# Autodesk Inventor assembly: Zed Kicker
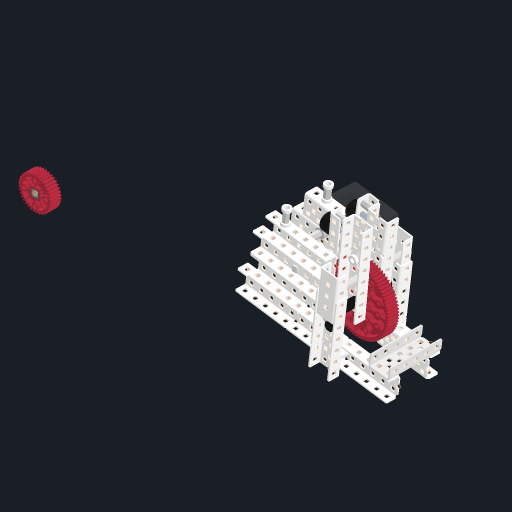
[picture p0: Inventor's stored thumbnail of the model, 512x512]
Saved by Autodesk Inventor 2023.2 (Build 272271030, 271C)
## iProperties
Created: 2024-02-14
Part Number: Zed Kicker
Document SubType Name: Assembly
Designer: Michael
Author: Michael
## Documents named in this file (35)
- C:\Users\black\OneDrive\Pictures\Documents\GitHub\New folder\2024-599Z\Cad\NEW Kicker\Zed Kicker.iam
- C:\Users\black\OneDrive\Pictures\Documents\GitHub\New folder\2024-599Z\Cad\Library\VEX-CAD-Inventor-1.4.0\Structure\C Channel\Aluminum 1x2x1\Alu C 1x2x1x15.ipt
- C:\Users\black\OneDrive\Pictures\Documents\GitHub\New folder\2024-599Z\Cad\Library\VEX-CAD-Inventor-1.4.0\Motion\Gears\HS Gear.iam
- C:\Users\black\OneDrive\Pictures\Documents\GitHub\New folder\2024-599Z\Cad\Library\VEX-CAD-Inventor-1.4.0\Structure\C Channel\Aluminum 1x2x1\Alu C 1x2x1x8.ipt
- C:\Users\black\OneDrive\Pictures\Documents\GitHub\New folder\2024-599Z\Cad\Library\VEX-CAD-Inventor-1.4.0\Structure\Standoff\Standoff .50.ipt
- C:\Users\black\OneDrive\Pictures\Documents\GitHub\New folder\2024-599Z\Cad\Library\VEX-CAD-Inventor-1.4.0\Structure\Standoff.ipt
- C:\Users\black\OneDrive\Pictures\Documents\GitHub\New folder\2024-599Z\Cad\Library\VEX-CAD-Inventor-1.4.0\Motion\Spacers\Spacer Nylon .313 OD\NSpacer .313 OD x .125.ipt
- C:\Users\black\OneDrive\Pictures\Documents\GitHub\New folder\2024-599Z\Cad\Library\VEX-CAD-Inventor-1.4.0\Motion\Spacers\Spacer Nylon .313 OD.ipt
- C:\Users\black\OneDrive\Pictures\Documents\GitHub\New folder\2024-599Z\Cad\Library\VEX-CAD-Inventor-1.4.0\Structure\Hardware\Rubber Bumper Threaded.ipt
- C:\Users\black\OneDrive\Pictures\Documents\GitHub\New folder\2024-599Z\Cad\Library\VEX-CAD-Inventor-1.4.0\Structure\C Channel\Aluminum 1x3x1 Half\Alu C Half 1x3x1x3.ipt
- C:\Users\black\OneDrive\Pictures\Documents\GitHub\New folder\2024-599Z\Cad\Library\VEX-CAD-Inventor-1.4.0\Motion\Shaft HS\HS Spacer\HSpacer .5000.ipt
- C:\Users\black\OneDrive\Pictures\Documents\GitHub\New folder\2024-599Z\Cad\Library\VEX-CAD-Inventor-1.4.0\Motion\Shaft HS\HS Spacer.ipt
- C:\Users\black\OneDrive\Pictures\Documents\GitHub\New folder\2024-599Z\Cad\Library\VEX-CAD-Inventor-1.4.0\Motion\Shaft HS\HS Spacer\HSpacer .1250.ipt
- C:\Users\black\OneDrive\Pictures\Documents\GitHub\New folder\2024-599Z\Cad\Library\VEX-CAD-Inventor-1.4.0\Motion\Shaft HS\HS Spacer\HSpacer .0625.ipt
- C:\Users\black\OneDrive\Pictures\Documents\GitHub\New folder\2024-599Z\Cad\Library\VEX-CAD-Inventor-1.4.0\Motion\Shaft HS\HS Spacer\HSpacer .2500.ipt
- C:\Users\black\OneDrive\Pictures\Documents\GitHub\New folder\2024-599Z\Cad\Library\VEX-CAD-Inventor-1.4.0\Structure\C Channel\Aluminum 1x2x1\Alu C 1x2x1x7.ipt
- C:\Users\black\OneDrive\Pictures\Documents\GitHub\New folder\2024-599Z\Cad\Library\VEX-CAD-Inventor-1.4.0\Motion\Gears\HS Gear\HS 36T Gear, No Insert.iam
- C:\Users\black\OneDrive\Pictures\Documents\GitHub\New folder\2024-599Z\Cad\Library\VEX-CAD-Inventor-1.4.0\Electronics\Motors with Screws\SteelM-StarS.iam
- C:\Users\black\OneDrive\Pictures\Documents\GitHub\New folder\2024-599Z\Cad\Library\VEX-CAD-Inventor-1.4.0\Electronics\Motors with Screws.iam
- C:\Users\black\OneDrive\Pictures\Documents\GitHub\New folder\2024-599Z\Cad\Library\VEX-CAD-Inventor-1.4.0\Structure\C Channel\Aluminum 1x2x1\Alu C 1x2x1x6.ipt
- C:\Users\black\OneDrive\Pictures\Documents\GitHub\New folder\2024-599Z\Cad\Library\VEX-CAD-Inventor-1.4.0\Shaft Collar (276-2010)\Shaft Collar (276-2010)_MIR1.ipt
- C:\Users\black\OneDrive\Pictures\Documents\GitHub\New folder\2024-599Z\Cad\Library\VEX-CAD-Inventor-1.4.0\Structure\Hardware\Nut Keps.ipt
- C:\Users\black\OneDrive\Pictures\Documents\GitHub\New folder\2024-599Z\Cad\Library\VEX-CAD-Inventor-1.4.0\Motion\Spacers\Spacer Nylon .313 OD\NSpacer .313 OD x .375.ipt
- C:\Users\black\OneDrive\Pictures\Documents\GitHub\New folder\2024-599Z\Cad\Library\VEX-CAD-Inventor-1.4.0\Motion\Spacers\Washer Teflon\TWasher .375 OD x .06250.ipt
- C:\Users\black\OneDrive\Pictures\Documents\GitHub\New folder\2024-599Z\Cad\Library\VEX-CAD-Inventor-1.4.0\Motion\Spacers\Washer Teflon.ipt
- C:\Users\black\OneDrive\Pictures\Documents\GitHub\New folder\2024-599Z\Cad\Library\VEX-CAD-Inventor-1.4.0\Motion\Spacers\Washer Teflon\TWasher .375 OD x .03125.ipt
- C:\Users\black\OneDrive\Pictures\Documents\GitHub\New folder\2024-599Z\Cad\Library\VEX-CAD-Inventor-1.4.0\Motion\Shaft HS\Shaft HS\Shaft HS 3.5 in.ipt
- C:\Users\black\OneDrive\Pictures\Documents\GitHub\New folder\2024-599Z\Cad\Library\VEX-CAD-Inventor-1.4.0\Motion\Shaft HS\Shaft HS.ipt
- C:\Users\black\OneDrive\Pictures\Documents\GitHub\New folder\2024-599Z\Cad\Library\VEX-CAD-Inventor-1.4.0\Structure\Gussets\C Channel Coupler.ipt
- C:\Users\black\OneDrive\Pictures\Documents\GitHub\New folder\2024-599Z\Cad\Library\VEX-CAD-Inventor-1.4.0\Motion\Shaft HS\HS Bearing Flat.ipt
- C:\Users\black\OneDrive\Pictures\Documents\GitHub\New folder\2024-599Z\Cad\Library\VEX-CAD-Inventor-1.4.0\Motion\Shaft HS\Shaft HS\Shaft HS 2.5 in.ipt
- C:\Users\black\OneDrive\Pictures\Documents\GitHub\New folder\2024-599Z\Cad\Library\VEX-CAD-Inventor-1.4.0\Motion\Gears\HS Gear\HS 12T Gear, No Insert.iam
- C:\Users\black\OneDrive\Pictures\Documents\GitHub\New folder\2024-599Z\Cad\Library\VEX-CAD-Inventor-1.4.0\Motion\Gears\HS Gear\HS 72T Gear, No Insert.iam
- C:\Users\black\OneDrive\Pictures\Documents\GitHub\New folder\2024-599Z\Cad\Library\VEX-CAD-Inventor-1.4.0\Motion\Spacers\Spacer Nylon .313 OD\NSpacer .313 OD x .500.ipt
- C:\Users\black\OneDrive\Pictures\Documents\GitHub\New folder\2024-599Z\Cad\Library\VEX-CAD-Inventor-1.4.0\Structure\C Channel\Aluminum 1x2x1\Alu C 1x2x1x5.ipt
## Components (61 placed, 27 different names)
1. Alu C 1x2x1x15:1 — Insert:81, Insert:82, Insert:86
2. Alu C 1x2x1x15:2 — Insert:77, Insert:78, Insert:85
3. Alu C 1x2x1x8:1 — Insert:75, Insert:76
4. Standoff .50:1
5. Standoff .50:2
6. Standoff .50:3
7. Standoff .50:4
8. Alu C 1x2x1x8:2 — Insert:87
9. NSpacer .313 OD x .125:1
10. Standoff .50:5
11. Standoff .50:6
12. NSpacer .313 OD x .125:2
13. Rubber Bumper Threaded:1
14. Rubber Bumper Threaded:2
15. Alu C Half 1x3x1x3:1
16. Alu C Half 1x3x1x3:2
17. HSpacer .5000:1
18. HSpacer .5000:2
19. HSpacer .1250:3
20. HSpacer .0625:4
21. HSpacer .2500:5
22. HSpacer .1250:6
23. HSpacer .2500:7
24. HSpacer .0625:8 — Insert:72
25. Alu C 1x2x1x7:1
26. Alu C 1x2x1x7:2
27. Alu C 1x2x1x7:3 — Insert:73
28. Alu C 1x2x1x7:4
29. HSpacer .1250:11 — Insert:73, Insert:74
30. SteelM-StarS:1 [sub-assembly]
31. NSpacer .313 OD x .125:3
32. Standoff .50:7
33. NSpacer .313 OD x .125:4
34. NSpacer .313 OD x .125:5
35. Standoff .50:8
36. NSpacer .313 OD x .125:6
37. Alu C 1x2x1x6:1
38. Alu C 1x2x1x6:2
39. Alu C 1x2x1x7:5 — Insert:83, Insert:84
40. Alu C 1x2x1x7:6 — Insert:72, Insert:79, Insert:80
41. Shaft Collar (276-2010)_MIR1:1
42. Nut Keps:1
43. Standoff .50:9
44. NSpacer .313 OD x .375:7
45. TWasher .375 OD x .06250:1
46. TWasher .375 OD x .03125:2
47. Shaft HS 3.5 in:1
48. C Channel Coupler:1
49. C Channel Coupler:2
50. Shaft HS 3.5 in:2
51. HS Bearing Flat:1
52. HS Bearing Flat:2
53. Shaft HS 2.5 in:3
54. HS 12T Gear, No Insert:2 [sub-assembly] — Insert:74
55. HS 72T Gear, No Insert:3 [sub-assembly] — Insert:75, Insert:76, Insert:87
56. NSpacer .313 OD x .500:8 — Insert:77, Insert:79
57. NSpacer .313 OD x .500:9 — Insert:78, Insert:80
58. NSpacer .313 OD x .500:10 — Insert:81, Insert:84
59. NSpacer .313 OD x .500:11 — Insert:82, Insert:83
60. HS 36T Gear, No Insert:4 [sub-assembly]
61. Alu C 1x2x1x5:1 — Insert:85, Insert:86
## Relationships (76: Insert 76)
- [Insert]: Alu C 1x2x1x8:1 ↔ Standoff .50:2
- [Insert]: Alu C 1x2x1x8:1 ↔ Standoff .50:1
- [Insert]: Standoff .50:3 ↔ Alu C 1x2x1x8:2
- [Insert]: Standoff .50:4 ↔ Alu C 1x2x1x8:2
- [Insert]: NSpacer .313 OD x .125:1 ↔ Standoff .50:5
- [Insert]: Alu C 1x2x1x8:1 ↔ Standoff .50:5
- [Insert]: Alu C 1x2x1x8:2 ↔ Standoff .50:6
- [Insert]: Standoff .50:6 ↔ NSpacer .313 OD x .125:2
- [Insert]: Standoff .50:1 ↔ Alu C Half 1x3x1x3:1
- [Insert]: Standoff .50:2 ↔ Alu C Half 1x3x1x3:1
- [Insert]: Rubber Bumper Threaded:2 ↔ Alu C Half 1x3x1x3:1
- [Insert]: Standoff .50:4 ↔ Alu C Half 1x3x1x3:2
- [Insert]: Standoff .50:3 ↔ Alu C Half 1x3x1x3:2
- [Insert]: Rubber Bumper Threaded:1 ↔ Alu C Half 1x3x1x3:2
- [Insert]: Alu C 1x2x1x8:1 ↔ HSpacer .5000:1
- [Insert]: Alu C 1x2x1x8:2 ↔ HSpacer .5000:2
- [Insert]: HSpacer .1250:3 ↔ HSpacer .0625:4
- [Insert]: HSpacer .5000:1 ↔ HSpacer .2500:5
- [Insert]: HSpacer .2500:5 ↔ HSpacer .1250:6
- [Insert]: HSpacer .1250:3 ↔ HSpacer .2500:7
- [Insert]: HSpacer .5000:2 ↔ HSpacer .2500:7
- [Insert]: HSpacer .1250:6 ↔ HSpacer .0625:8
- [Insert]: Alu C 1x2x1x15:1 ↔ Alu C 1x2x1x7:1
- [Insert]: Alu C 1x2x1x15:1 ↔ Alu C 1x2x1x7:1
- [Insert]: Alu C 1x2x1x7:1 ↔ Alu C 1x2x1x7:2
- [Insert]: Alu C 1x2x1x7:1 ↔ Alu C 1x2x1x7:2
- [Insert]: Alu C 1x2x1x7:3 ↔ Alu C 1x2x1x7:4
- [Insert]: Alu C 1x2x1x7:3 ↔ Alu C 1x2x1x7:4
- [Insert]: Alu C 1x2x1x15:2 ↔ Alu C 1x2x1x7:4
- [Insert]: Alu C 1x2x1x15:2 ↔ Alu C 1x2x1x7:4
- [Insert]: Alu C 1x2x1x7:2 ↔ SteelM-StarS:1
- [Insert]: Alu C 1x2x1x7:2 ↔ SteelM-StarS:1
- [Insert]: NSpacer .313 OD x .125:3 ↔ Standoff .50:7
- [Insert]: Standoff .50:7 ↔ NSpacer .313 OD x .125:4
- [Insert]: NSpacer .313 OD x .125:5 ↔ Standoff .50:8
- [Insert]: Standoff .50:8 ↔ NSpacer .313 OD x .125:6
- [Insert]: Alu C 1x2x1x7:3 ↔ Alu C 1x2x1x6:2
- [Insert]: Alu C 1x2x1x7:3 ↔ Alu C 1x2x1x6:2
- [Insert]: Alu C 1x2x1x7:2 ↔ Alu C 1x2x1x6:1
- [Insert]: Alu C 1x2x1x7:2 ↔ Alu C 1x2x1x6:1
- [Insert]: NSpacer .313 OD x .125:6 ↔ Alu C 1x2x1x6:1
- [Insert]: NSpacer .313 OD x .125:4 ↔ Alu C 1x2x1x6:2
- [Insert]: HSpacer .0625:4 ↔ Alu C 1x2x1x7:5
- [Insert]: Shaft Collar (276-2010)_MIR1:1 ↔ Nut Keps:1
- [Insert]: Shaft Collar (276-2010)_MIR1:1 ↔ Standoff .50:9
- [Insert]: Standoff .50:9 ↔ NSpacer .313 OD x .375:7
- [Insert]: NSpacer .313 OD x .375:7 ↔ TWasher .375 OD x .06250:1
- [Insert]: TWasher .375 OD x .06250:1 ↔ TWasher .375 OD x .03125:2
- [Insert]: Alu C 1x2x1x6:1 ↔ Nut Keps:1
- [Insert] (-54.61 mm): Alu C 1x2x1x8:1 ↔ Shaft HS 3.5 in:1
- [Insert]: Alu C 1x2x1x7:6 ↔ C Channel Coupler:2
- [Insert]: Alu C 1x2x1x7:6 ↔ C Channel Coupler:2
- [Insert]: Alu C 1x2x1x7:5 ↔ C Channel Coupler:1
- [Insert]: Alu C 1x2x1x7:5 ↔ C Channel Coupler:1
- [Insert]: Alu C 1x2x1x7:5 ↔ HS Bearing Flat:1
- [Insert]: Alu C 1x2x1x7:5 ↔ HS Bearing Flat:1
- [Insert]: Alu C 1x2x1x7:6 ↔ HS Bearing Flat:2
- [Insert]: Alu C 1x2x1x7:6 ↔ HS Bearing Flat:2
- [Insert] (-86.36 mm): Shaft HS 3.5 in:2 ↔ HS Bearing Flat:2
- [Insert] (-60.96 mm): Alu C 1x2x1x7:3 ↔ Shaft HS 2.5 in:3
- Insert:72: HSpacer .0625:8 ↔ Alu C 1x2x1x7:6
- Insert:73: Alu C 1x2x1x7:3 ↔ HSpacer .1250:11
- Insert:74: HSpacer .1250:11 ↔ HS 12T Gear, No Insert:2
- Insert:75: Alu C 1x2x1x8:1 ↔ HS 72T Gear, No Insert:3
- Insert:76: Alu C 1x2x1x8:1 ↔ HS 72T Gear, No Insert:3
- Insert:77: Alu C 1x2x1x15:2 ↔ NSpacer .313 OD x .500:8
- Insert:78: Alu C 1x2x1x15:2 ↔ NSpacer .313 OD x .500:9
- Insert:79: Alu C 1x2x1x7:6 ↔ NSpacer .313 OD x .500:8
- Insert:80: Alu C 1x2x1x7:6 ↔ NSpacer .313 OD x .500:9
- Insert:81: Alu C 1x2x1x15:1 ↔ NSpacer .313 OD x .500:10
- Insert:82: Alu C 1x2x1x15:1 ↔ NSpacer .313 OD x .500:11
- Insert:83: Alu C 1x2x1x7:5 ↔ NSpacer .313 OD x .500:11
- Insert:84: Alu C 1x2x1x7:5 ↔ NSpacer .313 OD x .500:10
- Insert:85: Alu C 1x2x1x15:2 ↔ Alu C 1x2x1x5:1
- Insert:86: Alu C 1x2x1x15:1 ↔ Alu C 1x2x1x5:1
- Insert:87: Alu C 1x2x1x8:2 ↔ HS 72T Gear, No Insert:3
## Named parameters: d164_d1232 = 0 mm, d167_d163 = 0 mm, d1321_d1235 = 0 mm
